# Autodesk Inventor assembly: Shooter_Assembly
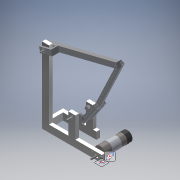
[picture p0: Inventor's stored thumbnail of the model, 180x180]
Saved by Autodesk Inventor 2019 (Build 230136000, 136)
## iProperties
Created: 2019-04-04
Part Number: Shooter_Assembly
Document SubType Name: Assembly
Designer: Delta
Author: Delta
## Documents named in this file (13)
- C:\Robotics\2019-20_CAD\offseason\random ideas\Shooter_Assembly.iam
- C:\Robotics\2019-20_CAD\offseason\random ideas\shooter.ipt
- shooter base.ipt
- C:\Robotics\2019-20_CAD\offseason\random ideas\Shooter_Stop.ipt
- C:\Robotics\COTSParts\Actobotics\585 parts\585384.ipt
- C:\Robotics\COTSParts\Actobotics\634 parts\634064.ipt
- C:\Robotics\COTSParts\Actobotics\634 parts\634068.25inDShaft2inLong.ipt
- C:\Robotics\2019-20_CAD\offseason\random ideas\Stop.ipt
- C:\Robotics\COTSParts\Actobotics\585 parts\585396MiniChannel7.7in.ipt
- C:\Robotics\COTSParts\Fasteners\nylon spacer 0.195ID 0.125.ipt
- C:\Robotics\2019-20_CAD\offseason\random ideas\shooter launch bar.ipt
- C:\Robotics\COTSParts\Bearings - AndyMark\Bearing 250 ID 500 OD flanged.ipt
- C:\Robotics\COTSParts\Motors\am-3102NeveRest20 (1).ipt
## Components (21 placed, 11 different names)
1. Shooter_Stop:1 — Insert:2, Insert:4, Mate:14, Mate:23
2. 585384:1 — Mate:4, Mate:22, Mate:23
3. shooter base:1 — Insert:9, Insert:10, Mate:14, Mate:18, Insert:14, Insert:15, Mate:26, Angle:1, Mate:27
4. 634064:1 — Insert:2, Mate:13
5. 634068.25inDShaft2inLong:1 — Mate:19, Mate:21, Flush:2
6. Stop:1 — Mate:3, Insert:13
7. 585384:2 — Mate:6, Mate:24, Mate:25
8. 585396MiniChannel7.7in:1 — Mate:8, Mate:9, Mate:10, Mate:11, Mate:17
9. Stop:2 — Insert:4, Mate:3
10. nylon spacer 0.195ID 0.125:1 — Mate:6, Mate:8, Mate:9, Mate:24
11. nylon spacer 0.195ID 0.125:2 — Mate:4, Mate:10, Mate:11, Mate:22
12. shooter launch bar:1 — Insert:7, Insert:8, Mate:17, Mate:18
13. Bearing 250 ID 500 OD flanged:3 — Insert:9, Mate:15
14. Bearing 250 ID 500 OD flanged:6 — Mate:19, Insert:14
15. Bearing 250 ID 500 OD flanged:7 — Insert:7
16. Bearing 250 ID 500 OD flanged:8 — Insert:10
17. Bearing 250 ID 500 OD flanged:9 — Mate:13, Insert:15
18. Bearing 250 ID 500 OD flanged:10 — Insert:8, Mate:16, Flush:1
19. 634068.25inDShaft2inLong:2 — Mate:15, Mate:16, Flush:1
20. Shooter_Stop:2 — Mate:21, Flush:2, Insert:13, Mate:25
21. am-3102NeveRest20 (1):1 — Mate:26, Angle:1, Mate:27
## Relationships (33: Mate 21, Insert 9, Flush 2, Angle 1)
- Insert:2: Shooter_Stop:1 ↔ 634064:1
- Insert:4: Shooter_Stop:1 ↔ Stop:2
- Mate:3: Stop:1 ↔ Stop:2
- Mate:4: 585384:1 ↔ nylon spacer 0.195ID 0.125:2
- Mate:6: 585384:2 ↔ nylon spacer 0.195ID 0.125:1
- Mate:8: 585396MiniChannel7.7in:1 ↔ nylon spacer 0.195ID 0.125:1
- Mate:9: 585396MiniChannel7.7in:1 ↔ nylon spacer 0.195ID 0.125:1
- Mate:10: 585396MiniChannel7.7in:1 ↔ nylon spacer 0.195ID 0.125:2
- Mate:11: 585396MiniChannel7.7in:1 ↔ nylon spacer 0.195ID 0.125:2
- Insert:7: shooter launch bar:1 ↔ Bearing 250 ID 500 OD flanged:7
- Insert:8: shooter launch bar:1 ↔ Bearing 250 ID 500 OD flanged:10
- Insert:9: shooter base:1 ↔ Bearing 250 ID 500 OD flanged:3
- Insert:10: shooter base:1 ↔ Bearing 250 ID 500 OD flanged:8
- Mate:13: 634064:1 ↔ Bearing 250 ID 500 OD flanged:9
- Mate:14 (0.127 mm): Shooter_Stop:1 ↔ shooter base:1
- Mate:15: Bearing 250 ID 500 OD flanged:3 ↔ 634068.25inDShaft2inLong:2
- Mate:16: Bearing 250 ID 500 OD flanged:10 ↔ 634068.25inDShaft2inLong:2
- Mate:17: 585396MiniChannel7.7in:1 ↔ shooter launch bar:1
- Mate:18 (1.27 mm): shooter base:1 ↔ shooter launch bar:1
- Flush:1: Bearing 250 ID 500 OD flanged:10 ↔ 634068.25inDShaft2inLong:2
- Mate:19: 634068.25inDShaft2inLong:1 ↔ Bearing 250 ID 500 OD flanged:6
- Mate:21: 634068.25inDShaft2inLong:1 ↔ Shooter_Stop:2
- Flush:2: 634068.25inDShaft2inLong:1 ↔ Shooter_Stop:2
- Insert:13: Stop:1 ↔ Shooter_Stop:2
- Mate:22: 585384:1 ↔ nylon spacer 0.195ID 0.125:2
- Mate:23: Shooter_Stop:1 ↔ 585384:1
- Mate:24: 585384:2 ↔ nylon spacer 0.195ID 0.125:1
- Mate:25: 585384:2 ↔ Shooter_Stop:2
- Insert:14: shooter base:1 ↔ Bearing 250 ID 500 OD flanged:6
- Insert:15: shooter base:1 ↔ Bearing 250 ID 500 OD flanged:9
- Mate:26: shooter base:1 ↔ am-3102NeveRest20 (1):1
- Angle:1 (180 deg): shooter base:1 ↔ am-3102NeveRest20 (1):1
- Mate:27: shooter base:1 ↔ am-3102NeveRest20 (1):1
